# Autodesk Inventor assembly: okragla mala napis
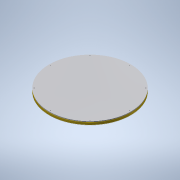
[picture p0: Inventor's stored thumbnail of the model, 180x180]
Saved by Autodesk Inventor 2021 (Build 250183000, 183)
## iProperties
Created: 2024-04-18
Part Number: okragla mala napis
Document SubType Name: Assembly
Designer: Michal
Author: Michal
## Documents named in this file (4)
- C:\Users\Michal\Documents\GitHub\PNW_PhotoBoothFrame_3D\okragla mala napis.iam
- C:\Users\Michal\Documents\GitHub\PNW_PhotoBoothFrame_3D\Kolo R600.ipt
- C:\Users\Michal\Documents\GitHub\PNW_PhotoBoothFrame_3D\płyta 6 biala okragla R600.ipt
- C:\Users\Michal\Documents\GitHub\PNW_PhotoBoothFrame_3D\materia okragly R600.ipt
## Components (3 placed, 3 different names)
1. Kolo R600:1 — Flush:26, Flush:27, Mate:35, Mate:37, Mate:38, Mate:39, Mate:40, Mate:41
2. płyta 6 biala okragla R600:1 — Mate:37, Mate:38, Mate:39
3. materia okragly R600:1 — Mate:40, Mate:41
## Relationships (8: Mate 6, Flush 2)
- Flush:26: Kolo R600:1
- Flush:27: Kolo R600:1
- Mate:35: Kolo R600:1
- Mate:37: Kolo R600:1 ↔ płyta 6 biala okragla R600:1
- Mate:38: Kolo R600:1 ↔ płyta 6 biala okragla R600:1
- Mate:39: Kolo R600:1 ↔ płyta 6 biala okragla R600:1
- Mate:40: Kolo R600:1 ↔ materia okragly R600:1
- Mate:41: Kolo R600:1 ↔ materia okragly R600:1
